# Autodesk Inventor assembly: Assembly1
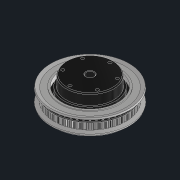
[picture p0: Inventor's stored thumbnail of the model, 180x180]
Saved by Autodesk Inventor 2022 (Build 260153000, 153)
## iProperties
Created: 2021-09-06
Part Number: Assembly1
Document SubType Name: Assembly
Designer: Yuta Kage
Author: Yuta Kage
## Documents named in this file (3)
- C:\Users\yuta0\Documents\GitHub\catchrobo_hardware\3d_print\Assembly1.iam
- C:\Users\yuta0\Documents\GitHub\catchrobo_hardware\assy-robot\base14.ipt
- C:\Users\yuta0\AppData\Local\Temp\Temp1_HTPB48S5M100-A-H59_Autodesk_Inventor_2020_20210906.zip\AIS2020\HTPB48S5M100-A-H59_b.ipt
## Components (2 placed, 2 different names)
1. base14:1 — メイト:1
2. HTPB48S5M100-A-H59_b:1 — メイト:1
## Relationships (1: Mate 1)
- メイト:1 [Mate]: base14:1 ↔ HTPB48S5M100-A-H59_b:1
